# Autodesk Inventor assembly: ASM IMU
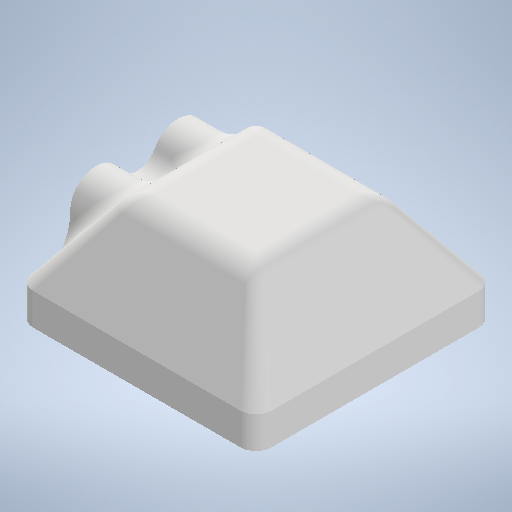
[picture p0: Inventor's stored thumbnail of the model, 512x512]
Saved by Autodesk Inventor 2025.2 (Build 292293000, 293)
## iProperties
Created: 2024-11-17
Part Number: ASM IMU
Document SubType Name: Assembly
Designer: tills
Author: tills
## Documents named in this file (5)
- C:\Users\tills\Desktop\Studium\Semester_3\Repositorys\Wearable-Health-Device\Inventor_AKTUELL\ASM IMU oben.iam
- C:\Users\tills\Desktop\Studium\Semester_3\Repositorys\Wearable-Health-Device\Inventor_AKTUELL\IMU_Base_T-Shirt.ipt
- C:\Users\tills\Desktop\Studium\Semester_3\Repositorys\Wearable-Health-Device\Inventor_AKTUELL\IMU_mount_baseplate.ipt
- C:\Users\tills\Desktop\Studium\Semester_3\Repositorys\Wearable-Health-Device\MPU6050 v2\MPU6050 v2.ipt
- C:\Users\tills\Desktop\Studium\Semester_3\Repositorys\Wearable-Health-Device\Inventor_AKTUELL\IMU_mount_cover_var_3.ipt
## Components (4 placed, 4 different names)
1. IMU_Base_T-Shirt:1 — Passend:1, Passend:2, Passend:3, Fluchtend:1, Fluchtend:2, Passend:9, Passend:10, Passend:11
2. IMU_mount_baseplate:1 — Passend:1, Passend:2, Passend:3, Passend:7, Passend:8
3. MPU6050 v2:1 — Passend:7, Passend:8
4. IMU_mount_cover_var_3:1 — Passend:9, Passend:10, Passend:11
## Relationships (10: Mate 8, Flush 2)
- Passend:1 [Mate] (3.5 mm): IMU_Base_T-Shirt:1 ↔ IMU_mount_baseplate:1
- Passend:2 [Mate] (3.5 mm): IMU_Base_T-Shirt:1 ↔ IMU_mount_baseplate:1
- Passend:3 [Mate]: IMU_Base_T-Shirt:1 ↔ IMU_mount_baseplate:1
- Fluchtend:1 [Flush] (-17 mm): IMU_Base_T-Shirt:1
- Fluchtend:2 [Flush] (-17 mm): IMU_Base_T-Shirt:1
- Passend:7 [Mate]: IMU_mount_baseplate:1 ↔ MPU6050 v2:1
- Passend:8 [Mate] (1 mm): IMU_mount_baseplate:1 ↔ MPU6050 v2:1
- Passend:9 [Mate]: IMU_Base_T-Shirt:1 ↔ IMU_mount_cover_var_3:1
- Passend:10 [Mate] (0.25 mm): IMU_Base_T-Shirt:1 ↔ IMU_mount_cover_var_3:1
- Passend:11 [Mate] (0.25 mm): IMU_Base_T-Shirt:1 ↔ IMU_mount_cover_var_3:1
